# Autodesk Inventor assembly: Wechselmechnanik
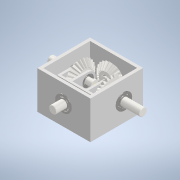
[picture p0: Inventor's stored thumbnail of the model, 180x180]
Saved by Autodesk Inventor 2021 (Build 250183000, 183)
## iProperties
Created: 2021-01-24
Part Number: Wechselmechnanik
Document SubType Name: Assembly
Designer: Jaro Machnow
Author: Jaro Machnow
## Documents named in this file (14)
- C:\Users\Jaro Machnow\Documents\Vault\Gruppen\Gruppe 2\Entwurf\Amphibienfahrzeug\Wechsel zwischen Land und Wasser\Mechanik_zum_Wechseln\Wechselmechnanik.iam
- C:\Users\Jaro Machnow\Documents\Vault\Gruppen\Gruppe 2\Entwurf\Amphibienfahrzeug\Wechsel zwischen Land und Wasser\Mechanik_zum_Wechseln\Wechselmechnanik\Konstruktions-Assistent\Wechsel_Kegelrad2_BG.iam
- C:\Users\Jaro Machnow\Documents\Vault\Gruppen\Gruppe 2\Entwurf\Amphibienfahrzeug\Wechsel zwischen Land und Wasser\Mechanik_zum_Wechseln\Wechsel_Welle_Antriebszahnrad.ipt
- C:\Users\Jaro Machnow\Documents\Vault\Gruppen\Gruppe 2\Entwurf\Amphibienfahrzeug\Wechsel zwischen Land und Wasser\Mechanik_zum_Wechseln\Wechsel_Welle-Schieben.ipt
- C:\Users\Jaro Machnow\Documents\Vault\Gruppen\Gruppe 2\Entwurf\Amphibienfahrzeug\Wechsel zwischen Land und Wasser\Mechanik_zum_Wechseln\Wechselmechnanik\Konstruktions-Assistent\Wechsel_Lager_Schieben.iam
- C:\Users\Jaro Machnow\Documents\Vault\Gruppen\Gruppe 2\Entwurf\Amphibienfahrzeug\Wechsel zwischen Land und Wasser\Mechanik_zum_Wechseln\Wechselmechnanik\Konstruktions-Assistent\Wechsel_Kegelrad1_BG.iam
- C:\Users\Jaro Machnow\Documents\Vault\Gruppen\Gruppe 2\Entwurf\Amphibienfahrzeug\Wechsel zwischen Land und Wasser\Wechselmechanik\Klappmechanismus\Klapp_Lager.iam
- C:\Users\Jaro Machnow\Documents\Vault\Gruppen\Gruppe 2\Entwurf\Amphibienfahrzeug\Wechsel zwischen Land und Wasser\Mechanik_zum_Wechseln\Wechsel_Hülle.ipt
- C:\Users\Jaro Machnow\Documents\Vault\Gruppen\Gruppe 2\Entwurf\Amphibienfahrzeug\Wechsel zwischen Land und Wasser\Mechanik_zum_Wechseln\Wechsel_Schiebeteil.ipt
- C:\Users\Jaro Machnow\Documents\Vault\Gruppen\Gruppe 2\Entwurf\Amphibienfahrzeug\Wechsel zwischen Land und Wasser\Mechanik_zum_Wechseln\Wechsel_Abstandsring.ipt
- C:\Users\Jaro Machnow\Documents\Vault\Gruppen\Gruppe 2\Entwurf\Amphibienfahrzeug\Wechsel zwischen Land und Wasser\Mechanik_zum_Wechseln\Wechsel_Zahnrad_fuer_Zahnstange.iam
- C:\Users\Jaro Machnow\Documents\Vault\Gruppen\Gruppe 2\Entwurf\Amphibienfahrzeug\Wechsel zwischen Land und Wasser\Mechanik_zum_Wechseln\Wechselmechnanik\Konstruktions-Assistent\Keilverbindung2.iam
- C:\Users\Jaro Machnow\Documents\Vault\Gruppen\Gruppe 2\Entwurf\Amphibienfahrzeug\Wechsel zwischen Land und Wasser\Mechanik_zum_Wechseln\Wechsel_Welle_Zahnrad_Zahnstange.ipt
- C:\Users\Jaro Machnow\Documents\Vault\Gruppen\Gruppe 2\Entwurf\Amphibienfahrzeug\Wechsel zwischen Land und Wasser\Mechanik_zum_Wechseln\Wechselmechnanik\Konstruktions-Assistent\Keilverbindung3.iam
## Components (25 placed, 8 different names)
1. Kegelräder:1 [sub-assembly] — Passend:2, Passend:18, Passend:20, Passend:61
2. Welle:1 — Passend:4, Winkel:2, Passend:22, Passend:53, Fluchtend:3, Winkel:6, Passend:59, Passend:62
3. Welle:1 — Passend:2, Passend:6, Passend:7, Passend:12, Passend:16, Passend:19, Passend:31, Passend:45, Passend:61
4. Lager:1 [sub-assembly] — Passend:7, Passend:17, Passend:47
5. Kegelräder:2 [sub-assembly] — Passend:4, Winkel:2, Passend:24, Passend:62
6. Lager:2 [sub-assembly] — Passend:6, Passend:48
7. Wechsel_Hülle:1 — Passend:12, Passend:27, Passend:29, Passend:30, Passend:40, Passend:41, Passend:42, Passend:51, Passend:52, Passend:54, Passend:55, Passend:56, Fluchtend:4, Passend:63
8. Lager:3 [sub-assembly] — Passend:27, Passend:28, Passend:52, Passend:53
9. Wechsel_Schiebeteil:1 — Passend:45, Passend:46, Passend:47, Passend:48, Passend:49, Passend:50, Passend:51
10. Wechsel_Abstandsring:1 — Passend:16, Passend:17, Passend:18
11. Wechsel_Abstandsring:2 — Passend:19, Passend:20
12. Wechsel_Zahnrad_fuer_Zahnstange:1 [sub-assembly] — Passend:54, Winkel:5
13. Keilverbindung:1 [sub-assembly] — Fluchtend:3, Winkel:6, Passend:59
14. Wechsel_Abstandsring:3 — Passend:22, Passend:24, Passend:28
15. Lager:4 [sub-assembly] — Passend:29, Passend:30, Passend:31
16. Kegelräder:3 [sub-assembly] — Passend:60
17. Welle:2 — Passend:40, Passend:43, Passend:46, Passend:60
18. Lager:5 [sub-assembly] — Passend:49
19. Lager:6 [sub-assembly] — Passend:50
20. Wechsel_Abstandsring:4
21. Wechsel_Abstandsring:5
22. Lager:7 [sub-assembly] — Passend:41, Passend:42, Passend:43
23. Lager:8 [sub-assembly] — Passend:55, Passend:56, Passend:57
24. Welle:1 — Passend:57, Fluchtend:2, Winkel:4, Passend:58, Winkel:5, Fluchtend:4
25. Keilverbindung:2 [sub-assembly] — Fluchtend:2, Winkel:4, Passend:58
## Relationships (55: Mate 48, Angle 4, Flush 3)
- Passend:2 [Mate]: Kegelräder:1 ↔ Welle:1
- Passend:4 [Mate]: Welle:1 ↔ Kegelräder:2
- Passend:6 [Mate]: Welle:1 ↔ Lager:2
- Passend:7 [Mate]: Welle:1 ↔ Lager:1
- Passend:12 [Mate]: Welle:1 ↔ Wechsel_Hülle:1
- Passend:16 [Mate]: Welle:1 ↔ Wechsel_Abstandsring:1
- Passend:17 [Mate]: Lager:1 ↔ Wechsel_Abstandsring:1
- Passend:18 [Mate]: Kegelräder:1 ↔ Wechsel_Abstandsring:1
- Passend:19 [Mate]: Welle:1 ↔ Wechsel_Abstandsring:2
- Passend:20 [Mate]: Kegelräder:1 ↔ Wechsel_Abstandsring:2
- Winkel:2 [Angle] (99.5917 deg): Welle:1 ↔ Kegelräder:2
- Passend:22 [Mate]: Welle:1 ↔ Wechsel_Abstandsring:3
- Passend:24 [Mate]: Kegelräder:2 ↔ Wechsel_Abstandsring:3
- Passend:27 [Mate]: Wechsel_Hülle:1 ↔ Lager:3
- Passend:28 [Mate]: Lager:3 ↔ Wechsel_Abstandsring:3
- Passend:29 [Mate]: Wechsel_Hülle:1 ↔ Lager:4
- Passend:30 [Mate]: Wechsel_Hülle:1 ↔ Lager:4
- Passend:31 [Mate]: Welle:1 ↔ Lager:4
- [Mate]: Kegelräder:3 ↔ Welle:2
- [Mate]: Welle:2 ↔ Lager:6
- [Mate]: Welle:2 ↔ Lager:5
- [Mate]: Welle:2 ↔ Wechsel_Abstandsring:4
- [Mate]: Lager:5 ↔ Wechsel_Abstandsring:4
- [Mate]: Kegelräder:3 ↔ Wechsel_Abstandsring:4
- [Mate]: Welle:2 ↔ Wechsel_Abstandsring:5
- [Mate]: Kegelräder:3 ↔ Wechsel_Abstandsring:5
- Passend:40 [Mate]: Wechsel_Hülle:1 ↔ Welle:2
- Passend:41 [Mate]: Wechsel_Hülle:1 ↔ Lager:7
- Passend:42 [Mate]: Wechsel_Hülle:1 ↔ Lager:7
- Passend:43 [Mate]: Welle:2 ↔ Lager:7
- Passend:45 [Mate]: Welle:1 ↔ Wechsel_Schiebeteil:1
- Passend:46 [Mate]: Wechsel_Schiebeteil:1 ↔ Welle:2
- Passend:47 [Mate]: Lager:1 ↔ Wechsel_Schiebeteil:1
- Passend:48 [Mate]: Lager:2 ↔ Wechsel_Schiebeteil:1
- Passend:49 [Mate]: Wechsel_Schiebeteil:1 ↔ Lager:5
- Passend:50 [Mate]: Wechsel_Schiebeteil:1 ↔ Lager:6
- Passend:51 [Mate]: Wechsel_Hülle:1 ↔ Wechsel_Schiebeteil:1
- Passend:52 [Mate]: Wechsel_Hülle:1 ↔ Lager:3
- Passend:53 [Mate]: Welle:1 ↔ Lager:3
- Passend:54 [Mate]: Wechsel_Hülle:1 ↔ Wechsel_Zahnrad_fuer_Zahnstange:1
- Passend:55 [Mate]: Wechsel_Hülle:1 ↔ Lager:8
- Passend:56 [Mate]: Wechsel_Hülle:1 ↔ Lager:8
- Passend:57 [Mate]: Lager:8 ↔ Welle:1
- Fluchtend:2 [Flush] (0.9339 mm): Welle:1 ↔ Keilverbindung:2
- Winkel:4 [Angle] (0 deg): Welle:1 ↔ Keilverbindung:2
- Passend:58 [Mate]: Welle:1 ↔ Keilverbindung:2
- Winkel:5 [Angle] (66.0073 deg): Wechsel_Zahnrad_fuer_Zahnstange:1 ↔ Welle:1
- Fluchtend:3 [Flush] (1.5781 mm): Welle:1 ↔ Keilverbindung:1
- Winkel:6 [Angle] (0 deg): Welle:1 ↔ Keilverbindung:1
- Passend:59 [Mate]: Welle:1 ↔ Keilverbindung:1
- Fluchtend:4 [Flush] (-1 mm): Wechsel_Hülle:1 ↔ Welle:1
- Passend:60 [Mate]: Kegelräder:3 ↔ Welle:2
- Passend:61 [Mate]: Kegelräder:1 ↔ Welle:1
- Passend:62 [Mate] (2 mm): Welle:1 ↔ Kegelräder:2
- Passend:63 [Mate]: Wechsel_Hülle:1
## Named parameters: d46_d28 = 0 mm, d47_d29 = 0 mm, d48_d25 = 0 mm, d49_d26 = 0 mm, d50_d27 = 0 mm, d51_d1 = 0 mm, d52_d11 = 0 mm, d53_d12 = 0 mm
